# Autodesk Inventor assembly: POM_T5_29
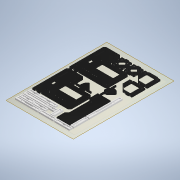
[picture p0: Inventor's stored thumbnail of the model, 180x180]
Saved by Autodesk Inventor 2020 (Build 240168000, 168)
## iProperties
Created: 2021-08-27
Part Number: POM_T5_29
Document SubType Name: Assembly
Designer: Masato
Author: Masato
## Documents named in this file (19)
- C:\Inventor\SUSTAINA-OP\Cam\POM_T5_29.iam
- C:\Inventor\SUSTAINA-OP\Cam\DisposableBoard.ipt
- C:\Inventor\SUSTAINA-OP\Jig\Cockpit_back_frame_Jig.ipt
- C:\Inventor\SUSTAINA-OP\Jig\Cockpit_battery_back_door_Jig.ipt
- C:\Inventor\SUSTAINA-OP\Jig\Cockpit_battery_bottom_frame_Jig_2.ipt
- C:\Inventor\SUSTAINA-OP\Jig\Cockpit_battery_bottom_frame_Jig.ipt
- C:\Inventor\SUSTAINA-OP\Jig\Cockpit_battery_front_frame_Jig.ipt
- C:\Inventor\SUSTAINA-OP\Jig\Cockpit_battery_front_frame_Jig_2.ipt
- C:\Inventor\SUSTAINA-OP\Jig\Cockpit_carrier_board_frame_Jig.ipt
- C:\Inventor\SUSTAINA-OP\Jig\Cockpit_front_frame_Jig.ipt
- C:\Inventor\SUSTAINA-OP\Jig\Cockpit_side_frame_Jig.ipt
- C:\Inventor\SUSTAINA-OP\Jig\BackLink_diagonal_Jig.ipt
- C:\Inventor\SUSTAINA-OP\Jig\Foot_root_block_Jig.ipt
- C:\Inventor\SUSTAINA-OP\Jig\Camera_side_frame_Jig.ipt
- C:\Inventor\SUSTAINA-OP\UpperBody\Cockpit\Cockpit_side_frame.ipt
- C:\Inventor\SUSTAINA-OP\UpperBody\Cockpit\Cockpit_battery_back_door.ipt
- C:\Inventor\SUSTAINA-OP\UpperBody\Head\Camera_side_frame.ipt
- C:\Inventor\SUSTAINA-OP\UpperBody\Arm\ForeArm_diagonal.ipt
- C:\Inventor\SUSTAINA-OP\UpperBody\Arm\UpperArm_diagonal.ipt
## Components (22 placed, 18 different names)
1. DisposableBoard:1 — メイト:2, メイト:1, フラッシュ:1, フラッシュ:2, メイト:4, フラッシュ:3, フラッシュ:4, メイト:5, メイト:6, メイト:9, メイト:10, メイト:13, メイト:15, メイト:16, メイト:18, メイト:21, メイト:25, メイト:27, メイト:29, メイト:30, メイト:33, メイト:36, メイト:39, メイト:40, メイト:43
2. Cockpit_battery_bottom_frame_Jig_2:1 — メイト:5, メイト:8, フラッシュ:6, メイト:50, メイト:53
3. Cockpit_battery_bottom_frame_Jig:1 — メイト:6, フラッシュ:5, メイト:7, メイト:8, メイト:49
4. Cockpit_back_frame_Jig:1 — メイト:4, フラッシュ:3, フラッシュ:4, フラッシュ:5, メイト:7, フラッシュ:6, フラッシュ:7, フラッシュ:10, メイト:23, フラッシュ:16
5. Cockpit_carrier_board_frame_Jig:1 — メイト:13, メイト:54, フラッシュ:19
6. Cockpit_battery_front_frame_Jig_2:1 — メイト:10, フラッシュ:8, メイト:12
7. Cockpit_battery_front_frame_Jig:1 — メイト:9, フラッシュ:7, フラッシュ:8, メイト:12, メイト:23, メイト:24
8. Cockpit_battery_back_door_Jig:1 — メイト:16, メイト:52, メイト:53, メイト:54, フラッシュ:19
9. Cockpit_side_frame_Jig:1 — メイト:18, フラッシュ:11, メイト:19, メイト:48
10. Cockpit_front_frame_Jig:1 — メイト:15, フラッシュ:10, フラッシュ:11, メイト:19, メイト:24, メイト:26, フラッシュ:14
11. BackLink_diagonal_Jig:1 — メイト:21, メイト:48, メイト:49
12. Foot_root_block_Jig:1 — メイト:25, メイト:26, フラッシュ:14, メイト:28, フラッシュ:15
13. Camera_side_frame_Jig:1 — メイト:27, メイト:28, フラッシュ:15, メイト:31
14. Cockpit_side_frame:1 — メイト:30, フラッシュ:17, メイト:32, メイト:41, メイト:46, メイト:47
15. Cockpit_side_frame:2 — メイト:29, メイト:31, フラッシュ:16, フラッシュ:17, メイト:32, メイト:35, メイト:37, メイト:38
16. Cockpit_battery_back_door:1 — メイト:33, メイト:35, メイト:42, メイト:50, メイト:52
17. Camera_side_frame:1 — メイト:36, メイト:37, メイト:38
18. Camera_side_frame:2 — メイト:40, メイト:41, メイト:42
19. ForeArm_diagonal:1 — メイト:43
20. ForeArm_diagonal:2 — メイト:51, フラッシュ:18
21. UpperArm_diagonal:1 — メイト:39, メイト:46, メイト:47
22. UpperArm_diagonal:2 — メイト:51, フラッシュ:18
## Component patterns: (2 elements, first: ForeArm_diagonal:1), (2 elements, first: UpperArm_diagonal:1)
## Relationships (61: Mate 45, Flush 16)
- メイト:2 [Mate]: DisposableBoard:1
- メイト:1 [Mate]: DisposableBoard:1
- フラッシュ:1 [Flush]: DisposableBoard:1
- フラッシュ:2 [Flush]: DisposableBoard:1
- メイト:4 [Mate]: DisposableBoard:1 ↔ Cockpit_back_frame_Jig:1
- フラッシュ:3 [Flush] (2.5 mm): DisposableBoard:1 ↔ Cockpit_back_frame_Jig:1
- フラッシュ:4 [Flush] (2 mm): DisposableBoard:1 ↔ Cockpit_back_frame_Jig:1
- メイト:5 [Mate]: DisposableBoard:1 ↔ Cockpit_battery_bottom_frame_Jig_2:1
- メイト:6 [Mate]: DisposableBoard:1 ↔ Cockpit_battery_bottom_frame_Jig:1
- フラッシュ:5 [Flush]: Cockpit_battery_bottom_frame_Jig:1 ↔ Cockpit_back_frame_Jig:1
- メイト:7 [Mate] (2.5 mm): Cockpit_battery_bottom_frame_Jig:1 ↔ Cockpit_back_frame_Jig:1
- メイト:8 [Mate] (2.5 mm): Cockpit_battery_bottom_frame_Jig_2:1 ↔ Cockpit_battery_bottom_frame_Jig:1
- フラッシュ:6 [Flush]: Cockpit_battery_bottom_frame_Jig_2:1 ↔ Cockpit_back_frame_Jig:1
- メイト:9 [Mate]: DisposableBoard:1 ↔ Cockpit_battery_front_frame_Jig:1
- メイト:10 [Mate]: DisposableBoard:1 ↔ Cockpit_battery_front_frame_Jig_2:1
- フラッシュ:7 [Flush]: Cockpit_back_frame_Jig:1 ↔ Cockpit_battery_front_frame_Jig:1
- フラッシュ:8 [Flush]: Cockpit_battery_front_frame_Jig_2:1 ↔ Cockpit_battery_front_frame_Jig:1
- メイト:12 [Mate] (2.1 mm): Cockpit_battery_front_frame_Jig_2:1 ↔ Cockpit_battery_front_frame_Jig:1
- メイト:13 [Mate]: DisposableBoard:1 ↔ Cockpit_carrier_board_frame_Jig:1
- メイト:15 [Mate]: DisposableBoard:1 ↔ Cockpit_front_frame_Jig:1
- メイト:16 [Mate]: DisposableBoard:1 ↔ Cockpit_battery_back_door_Jig:1
- フラッシュ:10 [Flush]: Cockpit_back_frame_Jig:1 ↔ Cockpit_front_frame_Jig:1
- メイト:18 [Mate]: DisposableBoard:1 ↔ Cockpit_side_frame_Jig:1
- フラッシュ:11 [Flush]: Cockpit_side_frame_Jig:1 ↔ Cockpit_front_frame_Jig:1
- メイト:19 [Mate] (2.5 mm): Cockpit_side_frame_Jig:1 ↔ Cockpit_front_frame_Jig:1
- メイト:21 [Mate]: DisposableBoard:1 ↔ BackLink_diagonal_Jig:1
- メイト:23 [Mate] (2.5 mm): Cockpit_back_frame_Jig:1 ↔ Cockpit_battery_front_frame_Jig:1
- メイト:24 [Mate] (2.5 mm): Cockpit_battery_front_frame_Jig:1 ↔ Cockpit_front_frame_Jig:1
- メイト:25 [Mate]: DisposableBoard:1 ↔ Foot_root_block_Jig:1
- メイト:26 [Mate] (2.5 mm): Cockpit_front_frame_Jig:1 ↔ Foot_root_block_Jig:1
- フラッシュ:14 [Flush]: Cockpit_front_frame_Jig:1 ↔ Foot_root_block_Jig:1
- メイト:27 [Mate]: DisposableBoard:1 ↔ Camera_side_frame_Jig:1
- メイト:28 [Mate] (2.5 mm): Foot_root_block_Jig:1 ↔ Camera_side_frame_Jig:1
- フラッシュ:15 [Flush]: Foot_root_block_Jig:1 ↔ Camera_side_frame_Jig:1
- メイト:29 [Mate]: DisposableBoard:1 ↔ Cockpit_side_frame:2
- メイト:30 [Mate]: DisposableBoard:1 ↔ Cockpit_side_frame:1
- メイト:31 [Mate] (2.5 mm): Camera_side_frame_Jig:1 ↔ Cockpit_side_frame:2
- フラッシュ:16 [Flush]: Cockpit_back_frame_Jig:1 ↔ Cockpit_side_frame:2
- フラッシュ:17 [Flush]: Cockpit_side_frame:1 ↔ Cockpit_side_frame:2
- メイト:32 [Mate] (2.5 mm): Cockpit_side_frame:1 ↔ Cockpit_side_frame:2
- メイト:33 [Mate]: DisposableBoard:1 ↔ Cockpit_battery_back_door:1
- メイト:35 [Mate] (2.5 mm): Cockpit_side_frame:2 ↔ Cockpit_battery_back_door:1
- メイト:36 [Mate]: DisposableBoard:1 ↔ Camera_side_frame:1
- メイト:37 [Mate] (2.5 mm): Cockpit_side_frame:2 ↔ Camera_side_frame:1
- メイト:38 [Mate] (2.5 mm): Cockpit_side_frame:2 ↔ Camera_side_frame:1
- メイト:39 [Mate]: DisposableBoard:1 ↔ UpperArm_diagonal:1
- メイト:40 [Mate]: DisposableBoard:1 ↔ Camera_side_frame:2
- メイト:41 [Mate] (2.5 mm): Cockpit_side_frame:1 ↔ Camera_side_frame:2
- メイト:42 [Mate] (2.5 mm): Cockpit_battery_back_door:1 ↔ Camera_side_frame:2
- メイト:43 [Mate]: DisposableBoard:1 ↔ ForeArm_diagonal:1
- メイト:46 [Mate] (2.5 mm): Cockpit_side_frame:1 ↔ UpperArm_diagonal:1
- メイト:47 [Mate] (2.5 mm): Cockpit_side_frame:1 ↔ UpperArm_diagonal:1
- メイト:48 [Mate] (2.1 mm): Cockpit_side_frame_Jig:1 ↔ BackLink_diagonal_Jig:1
- メイト:49 [Mate] (2.1 mm): Cockpit_battery_bottom_frame_Jig:1 ↔ BackLink_diagonal_Jig:1
- メイト:50 [Mate] (2.5 mm): Cockpit_battery_bottom_frame_Jig_2:1 ↔ Cockpit_battery_back_door:1
- メイト:51 [Mate] (2.5 mm): ForeArm_diagonal:2 ↔ UpperArm_diagonal:2
- フラッシュ:18 [Flush]: ForeArm_diagonal:2 ↔ UpperArm_diagonal:2
- メイト:52 [Mate] (2.5 mm): Cockpit_battery_back_door_Jig:1 ↔ Cockpit_battery_back_door:1
- メイト:53 [Mate] (2.5 mm): Cockpit_battery_bottom_frame_Jig_2:1 ↔ Cockpit_battery_back_door_Jig:1
- メイト:54 [Mate] (2.5 mm): Cockpit_carrier_board_frame_Jig:1 ↔ Cockpit_battery_back_door_Jig:1
- フラッシュ:19 [Flush]: Cockpit_carrier_board_frame_Jig:1 ↔ Cockpit_battery_back_door_Jig:1
